# Autodesk Inventor assembly: Ensamble Extr
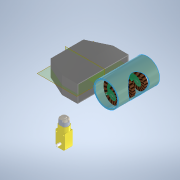
[picture p0: Inventor's stored thumbnail of the model, 180x180]
Saved by Autodesk Inventor 2020.3 (Build 243373000, 373)
## iProperties
Created: 2020-07-24
Part Number: Ensamble Extr
Document SubType Name: Assembly
Designer: juanp
Mass: 106.673 g
Surface Area: 956.147 cm^2
Volume: 101.984 cm^3
Density: 1.04598 g/cm^3
Author: juanp
## Documents named in this file (6)
- C:\Users\juanp\Desktop\Extr\Ensamble Extr.iam
- C:\Users\juanp\Desktop\Extr\Tornillo.ipt
- C:\Users\juanp\Desktop\Extr\Guía.ipt
- C:\Users\juanp\Desktop\ROBOCOL\Idea Final NAF\Motor\DC Motor Gearbox.iam
- C:\Users\juanp\Desktop\Extr\Eje.ipt
- C:\Users\juanp\Desktop\Extr\Tubo Interior.ipt
## Components (5 placed, 5 different names)
1. Tornillo:1 — Mate:13, Flush:1, Flush:2
2. Guía:1 — Mate:14
3. DC Motor Gearbox:1 [sub-assembly]
4. Eje:1 — Mate:13, Mate:14, Mate:15, Flush:2
5. Tubo Interior:1 — Mate:15, Flush:1
## Relationships (5: Mate 3, Flush 2)
- Mate:13: Tornillo:1 ↔ Eje:1
- Mate:14: Guía:1 ↔ Eje:1
- Mate:15: Eje:1 ↔ Tubo Interior:1
- Flush:1: Tornillo:1 ↔ Tubo Interior:1
- Flush:2: Tornillo:1 ↔ Eje:1
